# Autodesk Inventor assembly: Filament Runout Sensor Foot (1)
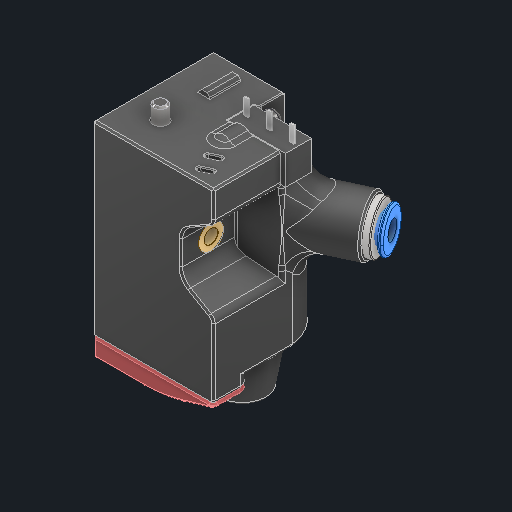
[picture p0: Inventor's stored thumbnail of the model, 512x512]
Saved by Autodesk Inventor 2025.1 (Build 291241020, 241B)
## iProperties
Created: 2025-05-09
Part Number: Filament Runout Sensor Foot (1)
Document SubType Name: Assembly
Designer: AdminForWorker
Title: Filament Runout Sensor Foot (1)
Author: AdminForWorker
## Documents named in this file (11)
- C:\Users\Joshua Eah\Documents\Voron 0.2\CAD\Master Assembly\Skirt\Filament Runout Sensor Foot.iam
- C:\Users\Joshua Eah\Documents\Voron 0.2\CAD\Master Assembly\Skirt\Rubber Foot.ipt
- C:\Users\Joshua Eah\Documents\Voron 0.2\CAD\Master Assembly\Hardware\M2x10 Self Tapper.ipt
- C:\Users\Joshua Eah\Documents\Voron 0.2\CAD\Master Assembly\Hardware\M3x40 BHCS.ipt
- C:\Users\Joshua Eah\Documents\Voron 0.2\CAD\Master Assembly\Hardware\M3x10 BHCS.ipt
- C:\Users\Joshua Eah\Documents\Voron 0.2\CAD\Master Assembly\Hardware\M3 Threaded Insert.ipt
- C:\Users\Joshua Eah\Documents\Voron 0.2\CAD\Master Assembly\Filament Runout Sensor Foot.ipt
- C:\Users\Joshua Eah\Documents\Voron 0.2\CAD\Master Assembly\ECAS04 Bowden Collet.ipt
- C:\Users\Joshua Eah\Documents\Voron 0.2\CAD\Master Assembly\Z Axis\Omron D2F Microswitch.ipt
- C:\Users\Joshua Eah\Documents\Voron 0.2\CAD\Master Assembly\Toolhead\Parts\Extruder\MR85 Bearing.ipt
- C:\Users\Joshua Eah\Documents\Voron 0.2\CAD\Master Assembly\Foot Accent Right.ipt
## Components (13 placed, 10 different names)
1. Filament Runout Sensor Foot:1 — Insert:4, Insert:5, Mate:1, Mate:2, Insert:6
2. Foot Accent Right:1 — Mate:2, Insert:6
3. M3 Threaded Insert:1
4. M3 Threaded Insert:2 — Insert:4
5. ECAS04 Bowden Collet:1
6. Omron D2F Microswitch:2 — Insert:5, Mate:1
7. MR85 Bearing:3
8. Rubber Foot:4
9. M2x10 Self Tapper:1
10. M2x10 Self Tapper:2
11. M2x10 Self Tapper:3
12. M3x40 BHCS:1
13. M3x10 BHCS:1
## Relationships (6: Insert 4, Mate 2)
- [Insert]: Omron D2F Microswitch:2 ↔ M2x10 Self Tapper:3
- Insert:4: Filament Runout Sensor Foot:1 ↔ M3 Threaded Insert:2
- Insert:5: Filament Runout Sensor Foot:1 ↔ Omron D2F Microswitch:2
- Mate:1: Filament Runout Sensor Foot:1 ↔ Omron D2F Microswitch:2
- Mate:2: Filament Runout Sensor Foot:1 ↔ Foot Accent Right:1
- Insert:6: Filament Runout Sensor Foot:1 ↔ Foot Accent Right:1
